# Autodesk Inventor assembly: SCR3D-6
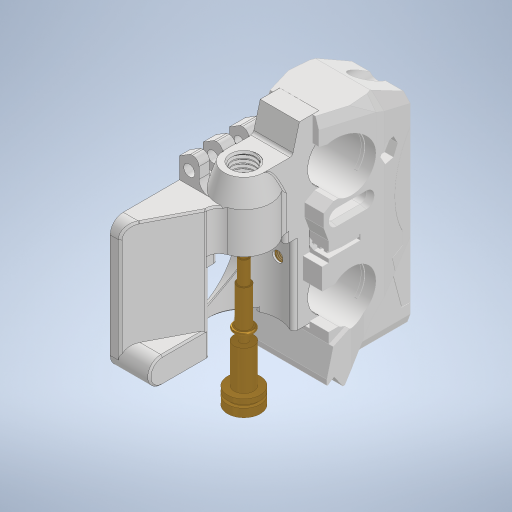
[picture p0: Inventor's stored thumbnail of the model, 512x512]
Saved by Autodesk Inventor 2023.1 (Build 271208000, 208)
## iProperties
Created: 2022-11-27
Part Number: SCR3D-6
Document SubType Name: Assembly
Designer: Frank
Author: Frank
## Documents named in this file (5)
- C:\Users\Frank\Desktop\SRC3D-6\SOURCE\SCR3D-6.iam
- C:\Users\Frank\Desktop\SRC3D-6\SOURCE\MINI-x-carriage.ipt
- C:\Users\Frank\Desktop\SRC3D-6\SOURCE\REVO-Micro Prusa Mini mount.ipt
- C:\Users\Frank\Desktop\SRC3D-6\SOURCE\Brass insert M3.ipt
- C:\Users\Frank\Desktop\SRC3D-6\SOURCE\REVO-Micro nozzle.ipt
## Components (7 placed, 4 different names)
1. MINI-x-carriage:1 — Mate:5, Mate:6, Mate:7
2. REVO-Micro Prusa Mini mount:1 — Mate:1, Mate:2, Mate:3, Mate:4, Flush:1, Flush:2, Flush:3, Flush:4, Flush:5, Flush:6, Angle:1, Angle:2
3. Brass insert M3:1 — Mate:1, Flush:1, Flush:5, Mate:5, Mate:7
4. Brass insert M3:2 — Mate:2, Flush:2, Flush:6, Mate:6
5. Brass insert M3:3 — Mate:3, Flush:3, Angle:1
6. Brass insert M3:4 — Mate:4, Flush:4, Angle:2
7. REVO-Micro nozzle:1
## Relationships (15: Mate 7, Flush 6, Angle 2)
- Mate:1: REVO-Micro Prusa Mini mount:1 ↔ Brass insert M3:1
- Mate:2: REVO-Micro Prusa Mini mount:1 ↔ Brass insert M3:2
- Mate:3: REVO-Micro Prusa Mini mount:1 ↔ Brass insert M3:3
- Mate:4: REVO-Micro Prusa Mini mount:1 ↔ Brass insert M3:4
- Flush:1: REVO-Micro Prusa Mini mount:1 ↔ Brass insert M3:1
- Flush:2: REVO-Micro Prusa Mini mount:1 ↔ Brass insert M3:2
- Flush:3: REVO-Micro Prusa Mini mount:1 ↔ Brass insert M3:3
- Flush:4: REVO-Micro Prusa Mini mount:1 ↔ Brass insert M3:4
- Flush:5: REVO-Micro Prusa Mini mount:1 ↔ Brass insert M3:1
- Flush:6: REVO-Micro Prusa Mini mount:1 ↔ Brass insert M3:2
- Angle:1 (0 deg): REVO-Micro Prusa Mini mount:1 ↔ Brass insert M3:3
- Angle:2 (0 deg): REVO-Micro Prusa Mini mount:1 ↔ Brass insert M3:4
- Mate:5: MINI-x-carriage:1 ↔ Brass insert M3:1
- Mate:6: MINI-x-carriage:1 ↔ Brass insert M3:2
- Mate:7: MINI-x-carriage:1 ↔ Brass insert M3:1
